# Autodesk Inventor assembly: Versaball
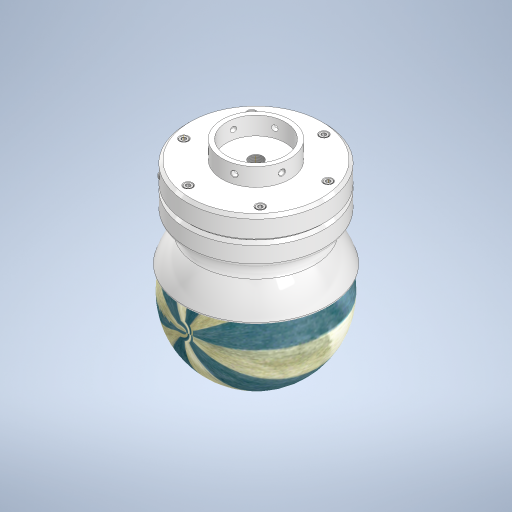
[picture p0: Inventor's stored thumbnail of the model, 512x512]
Saved by Autodesk Inventor 2023 (Build 270158030, 158C)
## iProperties
Created: 2022-09-15
Part Number: Versaball
Document SubType Name: Assembly
Designer: cjj5381
Mass: 1142.17 g
Surface Area: 3201.23 cm^2
Volume: 1266.29 cm^3
Density: 0.901982 g/cm^3
Author: cjj5381
## Documents named in this file (6)
- V:\Robtotics\Versaball.iam
- V:\Robtotics\Bottom.ipt
- V:\Robtotics\Versaball membrane.ipt
- V:\Robtotics\Top.ipt
- V:\Robtotics\Hardware\91290A254_NO THREADS_Black-Oxide Alloy Steel Socket Head Screw.ipt
- V:\Robtotics\Hardware\91375A825_NO THREADS_Alloy Steel Cup-Point Set Screw.ipt
## Components (10 placed, 5 different names)
1. Bottom:1 — Mate:1, Mate:2, Mate:3, Mate:4, Mate:5
2. Versaball membrane:1 — Mate:1, Mate:2
3. Top:1 — Mate:3, Mate:4, Mate:5, Mate:6, Mate:7, Mate:8, Mate:12, Mate:13
4. 91375A825_NO THREADS_Alloy Steel Cup-Point Set Screw:1 — Mate:13
5. 91290A254_NO THREADS_Black-Oxide Alloy Steel Socket Head Screw:7 — Mate:11, Mate:12
6. 91290A254_NO THREADS_Black-Oxide Alloy Steel Socket Head Screw:8
7. 91290A254_NO THREADS_Black-Oxide Alloy Steel Socket Head Screw:9
8. 91290A254_NO THREADS_Black-Oxide Alloy Steel Socket Head Screw:10
9. 91290A254_NO THREADS_Black-Oxide Alloy Steel Socket Head Screw:11
10. 91290A254_NO THREADS_Black-Oxide Alloy Steel Socket Head Screw:12
## Component patterns: (6 elements, first: 91290A254_NO THREADS_Black-Oxide Alloy Steel Socket Head Screw:7)
## Relationships (13: Mate 13)
- Mate:1: Bottom:1 ↔ Versaball membrane:1
- Mate:2: Bottom:1 ↔ Versaball membrane:1
- Mate:3: Bottom:1 ↔ Top:1
- Mate:4: Bottom:1 ↔ Top:1
- Mate:5: Bottom:1 ↔ Top:1
- Mate:6: Top:1
- Mate:7: Top:1
- Mate:8: Top:1
- Mate:9
- Mate:10
- Mate:11: 91290A254_NO THREADS_Black-Oxide Alloy Steel Socket Head Screw:7
- Mate:12: Top:1 ↔ 91290A254_NO THREADS_Black-Oxide Alloy Steel Socket Head Screw:7
- Mate:13: Top:1 ↔ 91375A825_NO THREADS_Alloy Steel Cup-Point Set Screw:1
